# Autodesk Inventor assembly: Ryan final assembley
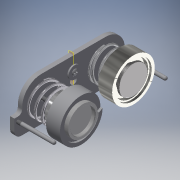
[picture p0: Inventor's stored thumbnail of the model, 180x180]
Saved by Autodesk Inventor 2017.1 (Build 211199000, 199)
## iProperties
Created: 2017-04-26
Part Number: Ryan final assembley
Document SubType Name: Assembly
Designer: 196918
Author: 196918
## Documents named in this file (15)
- C:\Users\196918\Desktop\Ryan final assembley.iam
- C:\Users\196918\Desktop\Base plate.ipt
- C:\Users\196918\Desktop\lever arm.ipt
- C:\Users\196918\Desktop\lower die 1 center.ipt
- C:\Users\196918\Desktop\lower die 1 outer ring.ipt
- C:\Users\196918\Desktop\Lower die 2 center.ipt
- C:\Users\196918\Desktop\Lower die 2 oweder ring.ipt
- C:\Users\196918\Desktop\lower die 2 spacer.ipt
- C:\Users\196918\Desktop\screw.ipt
- C:\Users\196918\Desktop\tiny screw.ipt
- C:\Users\196918\Desktop\Waher.ipt
- C:\Users\196918\Desktop\lever arm_MIR.ipt
- C:\Users\196918\Desktop\Bottom Die Spring 1.ipt
- C:\Users\196918\Desktop\Bottom Die Spring 1_MIR.ipt
- C:\Users\196918\Desktop\screw_MIR.ipt
## Components (14 placed, 14 different names)
1. Base plate:1 — Rigid:1, Mate:1, Angle:1, Mate:2, Angle:2, Rotational:1, Rotational:6, Rotational:8
2. lever arm:1 — Rigid:1
3. lower die 1 center:1 — Rotational:5
4. lower die 1 outer ring:1 — Rotational:4, Rotational:5
5. Lower die 2 center:1 — Rotational:3
6. Lower die 2 oweder ring:1 — Rotational:2, Rotational:3
7. lower die 2 spacer:1 — Rigid:2, Rotational:2
8. screw:1 — Rotational:8
9. tiny screw:1 — Rotational:6, Rotational:7
10. Waher:1 — Rotational:7
11. lever arm_MIR:1
12. Bottom Die Spring 1:1 — Rotational:1, Rotational:4
13. Bottom Die Spring 1_MIR:1 — Rigid:2
14. screw_MIR:1
## Relationships (15: RevoluteJoint 8, WeldJoint 2, Mate 2, Angle 2, Symmetry 1)
- Rigid:1 [WeldJoint]: Base plate:1 ↔ lever arm:1
- Mate:1: Base plate:1
- Angle:1 (0 deg): Base plate:1
- Mate:2: Base plate:1
- Angle:2 (0 deg): Base plate:1
- Symmetry:1
- Rotational:1 [RevoluteJoint]: Base plate:1 ↔ Bottom Die Spring 1:1
- Rigid:2 [WeldJoint]: lower die 2 spacer:1 ↔ Bottom Die Spring 1_MIR:1
- Rotational:2 [RevoluteJoint]: Lower die 2 oweder ring:1 ↔ lower die 2 spacer:1
- Rotational:3 [RevoluteJoint]: Lower die 2 center:1 ↔ Lower die 2 oweder ring:1
- Rotational:4 [RevoluteJoint]: lower die 1 outer ring:1 ↔ Bottom Die Spring 1:1
- Rotational:5 [RevoluteJoint]: lower die 1 center:1 ↔ lower die 1 outer ring:1
- Rotational:6 [RevoluteJoint]: Base plate:1 ↔ tiny screw:1
- Rotational:7 [RevoluteJoint]: tiny screw:1 ↔ Waher:1
- Rotational:8 [RevoluteJoint]: Base plate:1 ↔ screw:1
